# Autodesk Inventor assembly: MTLV-S01
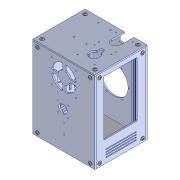
[picture p0: Inventor's stored thumbnail of the model, 180x180]
Saved by Autodesk Inventor 2020 (Build 240168000, 168)
## iProperties
Created: 2020-03-28
Part Number: MTLV-S01
Document SubType Name: Assembly
Designer: John K
Author: John K
## Documents named in this file (12)
- C:\GrabCAD\MTL Ventilator Design\MTLV\Subassemblies\MTLV-S01.iam
- C:\GrabCAD\MTL Ventilator Design\MTLV\Manufactured Parts\MTLV-M02.ipt
- C:\GrabCAD\MTL Ventilator Design\MTLV\Manufactured Parts\MTLV-M01 5537T501.ipt
- C:\GrabCAD\MTL Ventilator Design\MTLV\Manufactured Parts\MTLV-M03.ipt
- C:\GrabCAD\MTL Ventilator Design\MTLV\Manufactured Parts\MTLV-M04.ipt
- C:\GrabCAD\MTL Ventilator Design\MTLV\Manufactured Parts\MTLV-M05.ipt
- C:\GrabCAD\MTL Ventilator Design\MTLV\Manufactured Parts\MTLV-M06.ipt
- C:\GrabCAD\MTL Ventilator Design\MTLV\Manufactured Parts\MTLV-M07.ipt
- C:\GrabCAD\MTL Ventilator Design\MTLV\Commercial Parts\Misc\Bumper 9540K110.ipt
- C:\GrabCAD\MTL Ventilator Design\MTLV\Commercial Parts\Fasteners\M3x6mm Socket.ipt
- C:\GrabCAD\MTL Ventilator Design\MTLV\Commercial Parts\Fasteners\M5 T-Slot Fastener.ipt
- C:\GrabCAD\MTL Ventilator Design\MTLV\Commercial Parts\Fasteners\M5x10mm Flanged Button.ipt
## Components (58 placed, 11 different names)
1. MTLV-M01 5537T501:1 — Insert:1, Flush:2, Mate:4
2. MTLV-M01 5537T501:2 — Insert:2, Flush:2, Mate:1, Flush:4
3. MTLV-M01 5537T501:3 — Insert:3, Flush:1, Mate:2, Mate:5
4. MTLV-M01 5537T501:4 — Insert:4, Flush:1, Mate:3, Flush:8
5. MTLV-M02:1 — Insert:1, Insert:2, Insert:3, Insert:4, Flush:3, Flush:5, Flush:7, Flush:9, Insert:29, Insert:30, Insert:31, Insert:32
6. MTLV-M03:1 — Mate:1, Flush:3, Flush:4, Flush:6, Flush:12, Insert:37, Insert:38, Insert:61, Insert:62, Insert:63, Insert:64, Insert:77, Insert:78
7. MTLV-M04:1 — Mate:2, Flush:5, Flush:6, Flush:11, Insert:65, Insert:66, Insert:67, Insert:68, Insert:79, Insert:80, Insert:81, Insert:82
8. MTLV-M05:1 — Mate:3, Flush:7, Flush:8, Flush:10, Insert:69, Insert:70, Insert:71, Insert:72, Insert:83, Insert:84, Insert:85, Insert:86
9. MTLV-M06:1 — Mate:4, Flush:9, Flush:10, Insert:73, Insert:74, Insert:75, Insert:76, Insert:87, Insert:88, Insert:89, Insert:90
10. MTLV-M07:1 — Mate:5, Flush:11, Flush:12
11. M5x10mm Flanged Button:9 — Insert:61
12. M5x10mm Flanged Button:10 — Insert:62
13. M5x10mm Flanged Button:11 — Insert:63
14. M5x10mm Flanged Button:12 — Insert:64
15. M5x10mm Flanged Button:13 — Insert:65
16. M5x10mm Flanged Button:14 — Insert:66
17. M5x10mm Flanged Button:15 — Insert:67
18. M5x10mm Flanged Button:16 — Insert:68
19. M5x10mm Flanged Button:17 — Insert:69
20. M5x10mm Flanged Button:18 — Insert:70
21. M5x10mm Flanged Button:19 — Insert:71
22. M5x10mm Flanged Button:20 — Insert:72
23. M5x10mm Flanged Button:21 — Insert:73
24. M5x10mm Flanged Button:22 — Insert:74
25. M5x10mm Flanged Button:23 — Insert:75
26. M5x10mm Flanged Button:24 — Insert:76
27. M5x10mm Flanged Button:1
28. M5x10mm Flanged Button:2
29. M5x10mm Flanged Button:3
30. M5x10mm Flanged Button:4
31. M5x10mm Flanged Button:5
32. M5x10mm Flanged Button:6
33. M5x10mm Flanged Button:7
34. M5x10mm Flanged Button:8
35. M5 T-Slot Fastener:1 — Insert:37, Flush:19
36. M5 T-Slot Fastener:2 — Insert:38, Flush:19
37. M5 T-Slot Fastener:3 — Flush:18, Insert:77
38. M5 T-Slot Fastener:4 — Flush:18, Insert:78
39. M5 T-Slot Fastener:5 — Flush:17, Insert:79
40. M5 T-Slot Fastener:6 — Flush:17, Insert:80
41. M5 T-Slot Fastener:7 — Flush:16, Insert:81
42. M5 T-Slot Fastener:8 — Flush:16, Insert:82
43. M5 T-Slot Fastener:9 — Flush:15, Insert:83
44. M5 T-Slot Fastener:10 — Flush:15, Insert:84
45. M5 T-Slot Fastener:11 — Flush:14, Insert:85
46. M5 T-Slot Fastener:12 — Flush:14, Insert:86
47. M5 T-Slot Fastener:13 — Flush:13, Insert:87
48. M5 T-Slot Fastener:14 — Flush:13, Insert:88
49. M5 T-Slot Fastener:15 — Flush:20, Insert:89
50. M5 T-Slot Fastener:16 — Flush:20, Insert:90
51. Bumper 9540K110:1 — Insert:29, Insert:33
52. Bumper 9540K110:2 — Insert:30, Insert:36
53. Bumper 9540K110:3 — Insert:31, Insert:35
54. Bumper 9540K110:4 — Insert:32, Insert:34
55. M3x6mm Socket:1 — Insert:33
56. M3x6mm Socket:2 — Insert:34
57. M3x6mm Socket:3 — Insert:35
58. M3x6mm Socket:4 — Insert:36
## Relationships (77: Insert 52, Flush 20, Mate 5)
- Insert:1: MTLV-M01 5537T501:1 ↔ MTLV-M02:1
- Insert:2: MTLV-M01 5537T501:2 ↔ MTLV-M02:1
- Insert:3: MTLV-M01 5537T501:3 ↔ MTLV-M02:1
- Insert:4: MTLV-M01 5537T501:4 ↔ MTLV-M02:1
- Flush:1: MTLV-M01 5537T501:3 ↔ MTLV-M01 5537T501:4
- Flush:2: MTLV-M01 5537T501:1 ↔ MTLV-M01 5537T501:2
- Mate:1: MTLV-M01 5537T501:2 ↔ MTLV-M03:1
- Flush:3: MTLV-M02:1 ↔ MTLV-M03:1
- Flush:4: MTLV-M01 5537T501:2 ↔ MTLV-M03:1
- Mate:2: MTLV-M01 5537T501:3 ↔ MTLV-M04:1
- Flush:5: MTLV-M02:1 ↔ MTLV-M04:1
- Flush:6: MTLV-M03:1 ↔ MTLV-M04:1
- Mate:3: MTLV-M01 5537T501:4 ↔ MTLV-M05:1
- Flush:7: MTLV-M02:1 ↔ MTLV-M05:1
- Flush:8: MTLV-M01 5537T501:4 ↔ MTLV-M05:1
- Mate:4: MTLV-M01 5537T501:1 ↔ MTLV-M06:1
- Flush:9: MTLV-M02:1 ↔ MTLV-M06:1
- Flush:10: MTLV-M05:1 ↔ MTLV-M06:1
- Mate:5: MTLV-M01 5537T501:3 ↔ MTLV-M07:1
- Flush:11: MTLV-M04:1 ↔ MTLV-M07:1
- Flush:12: MTLV-M03:1 ↔ MTLV-M07:1
- Insert:29: MTLV-M02:1 ↔ Bumper 9540K110:1
- Insert:30: MTLV-M02:1 ↔ Bumper 9540K110:2
- Insert:31: MTLV-M02:1 ↔ Bumper 9540K110:3
- Insert:32: MTLV-M02:1 ↔ Bumper 9540K110:4
- Insert:33: Bumper 9540K110:1 ↔ M3x6mm Socket:1
- Insert:34: Bumper 9540K110:4 ↔ M3x6mm Socket:2
- Insert:35: Bumper 9540K110:3 ↔ M3x6mm Socket:3
- Insert:36: Bumper 9540K110:2 ↔ M3x6mm Socket:4
- Insert:37 (1.8 mm): MTLV-M03:1 ↔ M5 T-Slot Fastener:1
- Insert:38 (1.8 mm): MTLV-M03:1 ↔ M5 T-Slot Fastener:2
- Flush:13: M5 T-Slot Fastener:13 ↔ M5 T-Slot Fastener:14
- Flush:14: M5 T-Slot Fastener:11 ↔ M5 T-Slot Fastener:12
- Flush:15: M5 T-Slot Fastener:9 ↔ M5 T-Slot Fastener:10
- Flush:16: M5 T-Slot Fastener:7 ↔ M5 T-Slot Fastener:8
- Flush:17: M5 T-Slot Fastener:5 ↔ M5 T-Slot Fastener:6
- Flush:18: M5 T-Slot Fastener:3 ↔ M5 T-Slot Fastener:4
- Flush:19: M5 T-Slot Fastener:1 ↔ M5 T-Slot Fastener:2
- Flush:20: M5 T-Slot Fastener:15 ↔ M5 T-Slot Fastener:16
- [Insert]: MTLV-M02:1 ↔ M5x10mm Flanged Button:1
- [Insert]: MTLV-M02:1 ↔ M5x10mm Flanged Button:2
- [Insert]: MTLV-M02:1 ↔ M5x10mm Flanged Button:3
- [Insert]: MTLV-M02:1 ↔ M5x10mm Flanged Button:4
- [Insert]: MTLV-M07:1 ↔ M5x10mm Flanged Button:5
- [Insert]: MTLV-M07:1 ↔ M5x10mm Flanged Button:6
- [Insert]: MTLV-M07:1 ↔ M5x10mm Flanged Button:7
- [Insert]: MTLV-M07:1 ↔ M5x10mm Flanged Button:8
- Insert:61: MTLV-M03:1 ↔ M5x10mm Flanged Button:9
- Insert:62: MTLV-M03:1 ↔ M5x10mm Flanged Button:10
- Insert:63: MTLV-M03:1 ↔ M5x10mm Flanged Button:11
- Insert:64: MTLV-M03:1 ↔ M5x10mm Flanged Button:12
- Insert:65: MTLV-M04:1 ↔ M5x10mm Flanged Button:13
- Insert:66: MTLV-M04:1 ↔ M5x10mm Flanged Button:14
- Insert:67: MTLV-M04:1 ↔ M5x10mm Flanged Button:15
- Insert:68: MTLV-M04:1 ↔ M5x10mm Flanged Button:16
- Insert:69: MTLV-M05:1 ↔ M5x10mm Flanged Button:17
- Insert:70: MTLV-M05:1 ↔ M5x10mm Flanged Button:18
- Insert:71: MTLV-M05:1 ↔ M5x10mm Flanged Button:19
- Insert:72: MTLV-M05:1 ↔ M5x10mm Flanged Button:20
- Insert:73: MTLV-M06:1 ↔ M5x10mm Flanged Button:21
- Insert:74: MTLV-M06:1 ↔ M5x10mm Flanged Button:22
- Insert:75: MTLV-M06:1 ↔ M5x10mm Flanged Button:23
- Insert:76: MTLV-M06:1 ↔ M5x10mm Flanged Button:24
- Insert:77 (1.8 mm): MTLV-M03:1 ↔ M5 T-Slot Fastener:3
- Insert:78 (1.8 mm): MTLV-M03:1 ↔ M5 T-Slot Fastener:4
- Insert:79 (1.8 mm): MTLV-M04:1 ↔ M5 T-Slot Fastener:5
- Insert:80 (1.8 mm): MTLV-M04:1 ↔ M5 T-Slot Fastener:6
- Insert:81 (1.8 mm): MTLV-M04:1 ↔ M5 T-Slot Fastener:7
- Insert:82 (1.8 mm): MTLV-M04:1 ↔ M5 T-Slot Fastener:8
- Insert:83 (1.8 mm): MTLV-M05:1 ↔ M5 T-Slot Fastener:9
- Insert:84 (1.8 mm): MTLV-M05:1 ↔ M5 T-Slot Fastener:10
- Insert:85 (1.8 mm): MTLV-M05:1 ↔ M5 T-Slot Fastener:11
- Insert:86 (1.8 mm): MTLV-M05:1 ↔ M5 T-Slot Fastener:12
- Insert:87 (1.8 mm): MTLV-M06:1 ↔ M5 T-Slot Fastener:13
- Insert:88 (1.8 mm): MTLV-M06:1 ↔ M5 T-Slot Fastener:14
- Insert:89 (1.8 mm): MTLV-M06:1 ↔ M5 T-Slot Fastener:15
- Insert:90 (1.8 mm): MTLV-M06:1 ↔ M5 T-Slot Fastener:16
